# Autodesk Inventor assembly: Drive Train
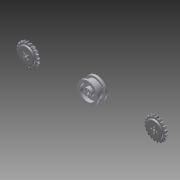
[picture p0: Inventor's stored thumbnail of the model, 180x180]
Saved by Autodesk Inventor 2015 (Build 190159000, 159)
## iProperties
Created: 2015-10-03
Part Number: Drive Train
Document SubType Name: Assembly
Designer: alhohbein
Author: alhohbein
## Documents named in this file (3)
- U:\Drive Train.iam
- U:\tetrix_736468_tt_wheel_2012.ipt
- U:\Tetrix tread sprocket.ipt
## Components (3 placed, 2 different names)
1. tetrix_736468_tt_wheel_2012:1 — Flush:1, Mate:1, DriveMe, Flush:2
2. Tetrix tread sprocket:1 — Flush:2, Mate:2, Mate:3, Flush:3
3. Tetrix tread sprocket:2 — Flush:3, Mate:4, Mate:5
## Relationships (9: Mate 5, Flush 3, Angle 1)
- Flush:1: tetrix_736468_tt_wheel_2012:1
- Mate:1: tetrix_736468_tt_wheel_2012:1
- DriveMe [Angle] (360 deg): tetrix_736468_tt_wheel_2012:1
- Flush:2 (-4.0005 mm): tetrix_736468_tt_wheel_2012:1 ↔ Tetrix tread sprocket:1
- Mate:2 (-3.175 mm): Tetrix tread sprocket:1
- Mate:3 (190.5 mm): Tetrix tread sprocket:1
- Flush:3: Tetrix tread sprocket:1 ↔ Tetrix tread sprocket:2
- Mate:4 (-3.175 mm): Tetrix tread sprocket:2
- Mate:5 (-190.5 mm): Tetrix tread sprocket:2
